# Autodesk Inventor assembly: motor mount - right
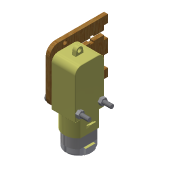
[picture p0: Inventor's stored thumbnail of the model, 180x180]
Saved by Autodesk Inventor 2016 (Build 200138000, 138)
## iProperties
Created: 2015-07-05
Part Number: motor mount - right
Document SubType Name: Assembly
Designer: Sebastian
Author: Sebastian
## Documents named in this file (5)
- J:\ERNIE\motor mount - right.iam
- J:\ERNIE\motor mount.ipt
- J:\ERNIE\motor.ipt
- J:\ERNIE\m3 30mm screw.ipt
- J:\ERNIE\3mm nut.ipt
## Components (6 placed, 4 different names)
1. motor mount:1 — Mate:1, Mate:2, Mate:3, Mate:5, Mate:6, Mate:7
2. m3 30mm screw:1 — Mate:4, Mate:5, Mate:8
3. m3 30mm screw:2 — Mate:6, Mate:7, Mate:9
4. 3mm nut:1 — Mate:8, Mate:10
5. 3mm nut:2 — Mate:9, Mate:11
6. motor:1 — Mate:1, Mate:2, Mate:3, Mate:4, Mate:10, Mate:11
## Relationships (11: Mate 11)
- Mate:1: motor mount:1 ↔ motor:1
- Mate:2: motor mount:1 ↔ motor:1
- Mate:3: motor mount:1 ↔ motor:1
- Mate:4: m3 30mm screw:1 ↔ motor:1
- Mate:5: motor mount:1 ↔ m3 30mm screw:1
- Mate:6: motor mount:1 ↔ m3 30mm screw:2
- Mate:7: motor mount:1 ↔ m3 30mm screw:2
- Mate:8: m3 30mm screw:1 ↔ 3mm nut:1
- Mate:9: m3 30mm screw:2 ↔ 3mm nut:2
- Mate:10: 3mm nut:1 ↔ motor:1
- Mate:11: 3mm nut:2 ↔ motor:1
